# Autodesk Inventor assembly: RT_ARM_A_001
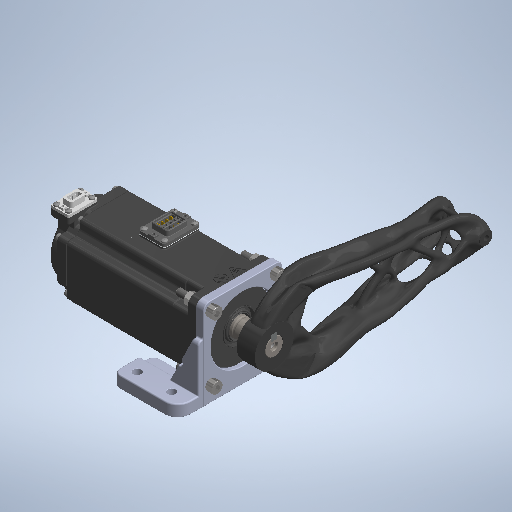
[picture p0: Inventor's stored thumbnail of the model, 512x512]
Saved by Autodesk Inventor 2025.3 (Build 293356000, 356)
## iProperties
Part Number: RT_ARM_A_001
Document SubType Name: Assembly
Designer: louis
Mass: 2815.38 g
Surface Area: 1885.74 cm^2
Volume: 559.711 cm^3
Density: 5.03006 g/cm^3
Author: louis
## Documents named in this file (12)
- C:\Users\louis\OneDrive\Desktop\R_Trident\02_CAD\04_Subassemblies\RT_ARM_A_001.iam
- C:\Users\louis\OneDrive\Desktop\R_Trident\02_CAD\01_Standard_Parts\A6M60-400H2B1-M17\A6M60-400H2B1-M17.iam
- C:\Users\louis\OneDrive\Desktop\R_Trident\02_CAD\01_Standard_Parts\ST-M4\ST-M4.ipt
- C:\Users\louis\OneDrive\Documents\Inventor\Content Center Files\R2025\en-US\ISO 4762(2)\ISO 4762 - M5 x 25ISO.ipt
- C:\Users\louis\OneDrive\Documents\Inventor\Content Center Files\R2025\en-US\ISO 4032(2)\ISO 4032 - M5 - ISO.ipt
- C:\Users\louis\OneDrive\Desktop\R_Trident\02_CAD\03_Parts_Custom\Study 2 - Structural Component - Outcome 6.ipt
- C:\Users\louis\OneDrive\Desktop\R_Trident\02_CAD\04_Subassemblies\RT_ARM_A_001\AIP\FEA\fff46vzts.fins
- C:\Users\louis\OneDrive\Desktop\R_Trident\02_CAD\04_Subassemblies\RT_ARM_A_001\AIP\FEA\fff46vzvk.fsat
- C:\Users\louis\OneDrive\Desktop\R_Trident\02_CAD\04_Subassemblies\RT_ARM_A_001\AIP\FEA\fff46vzvk.ftes
- C:\Users\louis\OneDrive\Desktop\R_Trident\02_CAD\04_Subassemblies\RT_ARM_A_001\AIP\FEA\fff46vzvk.fwiz
- C:\Users\louis\OneDrive\Desktop\R_Trident\02_CAD\04_Subassemblies\RT_ARM_A_001\AIP\FEA\fff46w0dc.fmsh
- C:\Users\louis\OneDrive\Desktop\R_Trident\02_CAD\04_Subassemblies\RT_ARM_A_001\AIP\FEA\fff46w0e8.fres
## Components (11 placed, 5 different names)
1. Study 2 - Structural Component - Outcome 6:1 — Mate:37, Mate:38, Flush:4
2. A6M60-400H2B1-M17:1 [sub-assembly] — Mate:15, Mate:16, Mate:17, Insert:5, Insert:6, Insert:7, Insert:8, Flush:1, Mate:19, Mate:37, Mate:38, Flush:4
3. ST-M4:1 — Mate:15, Mate:16, Mate:17, Mate:18, Insert:1, Insert:2, Insert:3, Insert:4
4. ISO 4762 M5 x 25:1 — Insert:1
5. ISO 4762 M5 x 25:2 — Insert:2
6. ISO 4762 M5 x 25:3 — Insert:3
7. ISO 4762 M5 x 25:4 — Insert:4
8. ISO 4032 M5:1 — Insert:5
9. ISO 4032 M5:2 — Insert:6
10. ISO 4032 M5:3 — Insert:7
11. ISO 4032 M5:4 — Insert:8
## Relationships (17: Insert 8, Mate 7, Flush 2)
- Mate:15: A6M60-400H2B1-M17:1 ↔ ST-M4:1
- Mate:16: A6M60-400H2B1-M17:1 ↔ ST-M4:1
- Mate:17: A6M60-400H2B1-M17:1 ↔ ST-M4:1
- Mate:18: ST-M4:1
- Insert:1: ST-M4:1 ↔ ISO 4762 M5 x 25:1
- Insert:2: ST-M4:1 ↔ ISO 4762 M5 x 25:2
- Insert:3: ST-M4:1 ↔ ISO 4762 M5 x 25:3
- Insert:4: ST-M4:1 ↔ ISO 4762 M5 x 25:4
- Insert:5: A6M60-400H2B1-M17:1 ↔ ISO 4032 M5:1
- Insert:6: A6M60-400H2B1-M17:1 ↔ ISO 4032 M5:2
- Insert:7: A6M60-400H2B1-M17:1 ↔ ISO 4032 M5:3
- Insert:8: A6M60-400H2B1-M17:1 ↔ ISO 4032 M5:4
- Flush:1: A6M60-400H2B1-M17:1
- Mate:19: A6M60-400H2B1-M17:1
- Mate:37: Study 2 - Structural Component - Outcome 6:1 ↔ A6M60-400H2B1-M17:1
- Mate:38: Study 2 - Structural Component - Outcome 6:1 ↔ A6M60-400H2B1-M17:1
- Flush:4: Study 2 - Structural Component - Outcome 6:1 ↔ A6M60-400H2B1-M17:1
## Named parameters: sa_0 = 40000, sa_1 = 100000
note: some values were not read from the file. Shown as the stored number, unit unknown: "sa_0", "sa_1".
